# Autodesk Inventor assembly: Quad correct axis
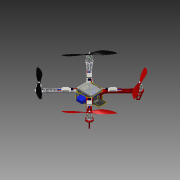
[picture p0: Inventor's stored thumbnail of the model, 180x180]
Saved by Autodesk Inventor 2015 (Build 190159000, 159)
## iProperties
Created: 2015-06-20
Part Number: Quad correct axis
Document SubType Name: Assembly
Designer: Benjamin
Mass: 1060.83 g
Surface Area: 3106.6 cm^2
Volume: 458.713 cm^3
Density: 2.31262 g/cm^3
Author: Benjamin
## Documents named in this file (2)
- C:\Users\Lauszus\Dropbox\kristian\Kristian\Quad correct axis.iam
- C:\Users\Lauszus\Dropbox\Kristian\Kristian\Quad wrong axis.iam
## Components (1 placed, 1 different names)
1. Quad wrong axis:1 [sub-assembly] — Mate:1, Mate:2
## Relationships (2: Mate 2)
- Mate:1: Quad wrong axis:1
- Mate:2: Quad wrong axis:1
